# Autodesk Inventor assembly: motor test assy
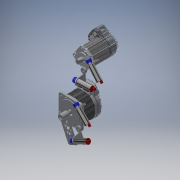
[picture p0: Inventor's stored thumbnail of the model, 180x180]
Saved by Autodesk Inventor 2018.2 (Build 222227000, 227)
## iProperties
Created: 2018-03-04
Part Number: motor test assy
Document SubType Name: Assembly
Designer: torba
Author: torba
## Documents named in this file (8)
- C:\Users\torba\OneDrive\Documents\Inventor\Plasma 5x10\motor test assy.iam
- C:\Users\torba\OneDrive\Documents\Inventor\Plasma 5x10\CPM-341x\CPM-_ _ _ _ - 3411_-LS.ipt
- C:\Users\torba\OneDrive\Documents\Inventor\Plasma 5x10\Limit Switch.ipt
- C:\Users\torba\OneDrive\Documents\Inventor\Plasma 5x10\Test Mount Limit Servo.ipt
- C:\Users\torba\OneDrive\Documents\Inventor\Plasma 5x10\motor test flapper.ipt
- C:\Users\torba\OneDrive\Documents\Inventor\Plasma 5x10\CPM-232x\CPM-_ _ _ _ -2321_-LS.ipt
- C:\Users\torba\OneDrive\Documents\Inventor\Plasma 5x10\Test Mount Limit Servo nema23.ipt
- C:\Users\torba\OneDrive\Documents\Inventor\Plasma 5x10\motor test flapper nema23 v2.ipt
## Components (12 placed, 7 different names)
1. CPM-_ _ _ _ - 3411_-LS:1 — Mate:1, Mate:2, Mate:3, Mate:4, Angle:2, Mate:7, Flush:3
2. Limit Switch:1 — Mate:5, Flush:2
3. Test Mount Limit Servo:1 — Mate:1, Mate:3, Mate:6, Flush:1
4. Test Mount Limit Servo:2 — Mate:2, Mate:4, Angle:2, Mate:5, Flush:2
5. Limit Switch:2 — Mate:6, Flush:1, Mate:8
6. motor test flapper:1 — Mate:7, Mate:8
7. CPM-_ _ _ _ -2321_-LS:1 — Flush:3, Mate:9, Mate:10, Mate:11, Mate:12, Mate:16
8. Limit Switch:3 — Mate:14, Flush:5
9. Limit Switch:4 — Mate:13, Flush:4, Mate:15
10. Test Mount Limit Servo nema23:1 — Mate:9, Mate:11, Mate:13, Flush:4
11. Test Mount Limit Servo nema23:2 — Mate:10, Mate:12, Mate:14, Flush:5
12. motor test flapper nema23 v2:1 — Mate:15, Mate:16
## Relationships (22: Mate 16, Flush 5, Angle 1)
- Mate:1: CPM-_ _ _ _ - 3411_-LS:1 ↔ Test Mount Limit Servo:1
- Mate:2: CPM-_ _ _ _ - 3411_-LS:1 ↔ Test Mount Limit Servo:2
- Mate:3: CPM-_ _ _ _ - 3411_-LS:1 ↔ Test Mount Limit Servo:1
- Mate:4: CPM-_ _ _ _ - 3411_-LS:1 ↔ Test Mount Limit Servo:2
- Angle:2 (45 deg): CPM-_ _ _ _ - 3411_-LS:1 ↔ Test Mount Limit Servo:2
- Mate:5: Limit Switch:1 ↔ Test Mount Limit Servo:2
- Mate:6: Test Mount Limit Servo:1 ↔ Limit Switch:2
- Flush:1 (-12.7 mm): Test Mount Limit Servo:1 ↔ Limit Switch:2
- Flush:2 (-12.7 mm): Limit Switch:1 ↔ Test Mount Limit Servo:2
- Mate:7: CPM-_ _ _ _ - 3411_-LS:1 ↔ motor test flapper:1
- Mate:8: Limit Switch:2 ↔ motor test flapper:1
- Flush:3: CPM-_ _ _ _ - 3411_-LS:1 ↔ CPM-_ _ _ _ -2321_-LS:1
- Mate:9: CPM-_ _ _ _ -2321_-LS:1 ↔ Test Mount Limit Servo nema23:1
- Mate:10: CPM-_ _ _ _ -2321_-LS:1 ↔ Test Mount Limit Servo nema23:2
- Mate:11: CPM-_ _ _ _ -2321_-LS:1 ↔ Test Mount Limit Servo nema23:1
- Mate:12: CPM-_ _ _ _ -2321_-LS:1 ↔ Test Mount Limit Servo nema23:2
- Mate:13: Limit Switch:4 ↔ Test Mount Limit Servo nema23:1
- Mate:14: Limit Switch:3 ↔ Test Mount Limit Servo nema23:2
- Flush:4 (-12.7 mm): Limit Switch:4 ↔ Test Mount Limit Servo nema23:1
- Flush:5 (12.7 mm): Limit Switch:3 ↔ Test Mount Limit Servo nema23:2
- Mate:15: Limit Switch:4 ↔ motor test flapper nema23 v2:1
- Mate:16: CPM-_ _ _ _ -2321_-LS:1 ↔ motor test flapper nema23 v2:1
